# Autodesk Inventor assembly: sch40conduit
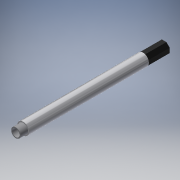
[picture p0: Inventor's stored thumbnail of the model, 180x180]
Saved by Autodesk Inventor 2017 (Build 210142000, 142)
## iProperties
Created: 2018-11-30
Part Number: sch40conduit
Document SubType Name: Assembly
Designer: ddeboer
Author: ddeboer
## Documents named in this file (4)
- C:\Users\ddeboer\Desktop\sch40_conduit\sch40conduit.iam
- C:\Users\ddeboer\Desktop\sch40_conduit\conduit_endcap.ipt
- C:\Users\ddeboer\Desktop\sch40_conduit\outer_sheath.ipt
- C:\Users\ddeboer\Desktop\sch40_conduit\inner_assy.iam
## Components (3 placed, 3 different names)
1. conduit_endcap:1 — Insert:1, Insert:2
2. outer_sheath:1 — Insert:1
3. inner_assy:1 [sub-assembly] — Insert:2
## Relationships (2: Insert 2)
- Insert:1 (-400 mm): conduit_endcap:1 ↔ outer_sheath:1
- Insert:2: conduit_endcap:1 ↔ inner_assy:1
